# Autodesk Inventor assembly: Fuel Grain
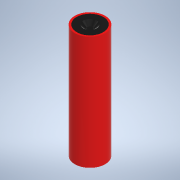
[picture p0: Inventor's stored thumbnail of the model, 180x180]
Saved by Autodesk Inventor 2021 (Build 250183000, 183)
## iProperties
Created: 2021-08-22
Part Number: Fuel Grain
Document SubType Name: Assembly
Designer: Alex Clay
Author: Alex Clay
## Documents named in this file (3)
- C:\Users\alexc\Embry-Riddle Aeronautical University\Kingsberry, Kyle A. - Odyssey\ODSY-ASSY V3\ODSY-0003 V0\Fuel Grain.iam
- C:\Users\alexc\Embry-Riddle Aeronautical University\Kingsberry, Kyle A. - Odyssey\ODSY-ASSY V3\ODSY-0003 V0\Phenolic Tube.ipt
- C:\Users\alexc\Embry-Riddle Aeronautical University\Kingsberry, Kyle A. - Odyssey\ODSY-ASSY V3\ODSY-0003 V0\Fuel Grain.ipt
## Components (2 placed, 2 different names)
1. Phenolic Tube:1 — Mate:1, Mate:2, Mate:3, Mate:4, Flush:2
2. Fuel Grain:1 — Mate:4, Flush:1, Flush:2
## Relationships (6: Mate 4, Flush 2)
- Mate:1: Phenolic Tube:1
- Mate:2: Phenolic Tube:1
- Mate:3: Phenolic Tube:1
- Mate:4: Phenolic Tube:1 ↔ Fuel Grain:1
- Flush:1: Fuel Grain:1
- Flush:2: Phenolic Tube:1 ↔ Fuel Grain:1
